# Autodesk Inventor assembly: drive with fourbar linkage
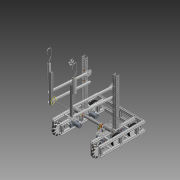
[picture p0: Inventor's stored thumbnail of the model, 180x180]
Saved by Autodesk Inventor 2013 (Build 170138000, 138)
## iProperties
Created: 2013-12-21
Part Number: drive with fourbar linkage
Document SubType Name: Assembly
Designer: kahohbein
Author: kahohbein
## Documents named in this file (22)
- C:\Users\nojessen\Documents\GitHub\2013-2014_BlockParty\CAD\wimp with full update.iam
- C:\Users\nojessen\Documents\GitHub\2013-2014_BlockParty\CAD\Drive\Final Drive Complete\Driveopen2.iam
- C:\Users\nojessen\Documents\GitHub\2013-2014_BlockParty\CAD\COTSParts\Tetrix\Tetrix flat plate.ipt
- C:\Users\nojessen\Documents\GitHub\2013-2014_BlockParty\CAD\COTSParts\Tetrix\Tetrix channel 32mm.ipt
- C:\Users\nojessen\Documents\GitHub\2013-2014_BlockParty\CAD\COTSParts\Tetrix\Bronze bushing.ipt
- C:\Users\nojessen\Documents\GitHub\2013-2014_BlockParty\CAD\COTSParts\Tetrix\Tetrix motor mount.ipt
- C:\Users\nojessen\Documents\GitHub\2013-2014_BlockParty\CAD\Lift\MK3\hook prototype.ipt
- C:\Users\nojessen\Documents\GitHub\2013-2014_BlockParty\CAD\Lift\Bosch 20x20 modified.ipt
- C:\Users\nojessen\Documents\GitHub\2013-2014_BlockParty\CAD\four bar linkage\custom Box Aluminum.ipt
- C:\Users\nojessen\Documents\GitHub\2013-2014_BlockParty\CAD\four bar linkage\custom bosch 8in.ipt
- C:\Users\nojessen\Documents\GitHub\2013-2014_BlockParty\CAD\COTSParts\Tetrix\Tetrix Channel 416mm.ipt
- C:\Users\nojessen\Documents\GitHub\2013-2014_BlockParty\CAD\COTSParts\Tetrix\Tetrix Channel 416mm_CPY.ipt
- C:\Users\nojessen\Documents\GitHub\2013-2014_BlockParty\CAD\COTSParts\Tetrix\Tetrix Hub - axle.ipt
- C:\Users\nojessen\Documents\GitHub\2013-2014_BlockParty\CAD\COTSParts\Tetrix\Tetrix sprocket 24T.ipt
- C:\Users\nojessen\Documents\GitHub\2013-2014_BlockParty\CAD\Lift\MK4\Winch MK4.iam
- C:\Users\nojessen\Documents\GitHub\2013-2014_BlockParty\CAD\COTSParts\Fasteners\4-40 SHCS x125.ipt
- C:\Users\nojessen\Documents\GitHub\2013-2014_BlockParty\CAD\Lift\MK4\ratchet stop mk 2.ipt
- C:\Users\nojessen\Documents\GitHub\2013-2014_BlockParty\CAD\Lift\MK4\Tetrix channel 32mm modified.ipt
- C:\Users\nojessen\Documents\GitHub\2013-2014_BlockParty\CAD\Pick-up Blocks\axle.ipt
- C:\Users\nojessen\Documents\GitHub\2013-2014_BlockParty\CAD\COTSParts\Tetrix\Tetrix sprocket 16T_MIR2.ipt
- C:\Users\nojessen\Documents\GitHub\2013-2014_BlockParty\CAD\COTSParts\Tetrix\Tetrix Hub - axle_MIR2.ipt
- C:\Users\nojessen\Documents\GitHub\2013-2014_BlockParty\CAD\COTSParts\Bosch Extrusion\Gusset 20x20 w screws.ipt
## Components (43 placed, 21 different names)
1. Driveopen2:1 [sub-assembly] — Mate:1, Mate:2, Mate:3, Mate:4, Mate:5, Mate:6
2. Tetrix flat plate:1 — Mate:2, Mate:3, Mate:4, Mate:15, Mate:16, Mate:110, Flush:10, Mate:184, Mate:191, Mate:192, Mate:193, Mate:201, Mate:202
3. Tetrix flat plate:2 — Mate:1, Mate:5, Mate:6, Mate:11, Mate:12, Mate:100, Flush:8, Mate:176, Mate:194, Mate:195, Mate:196, Mate:199, Mate:200
4. Tetrix channel 32mm:1 — Mate:15, Mate:16, Flush:9, Mate:111, Flush:10
5. Tetrix channel 32mm:2 — Mate:11, Mate:12, Mate:101, Flush:7, Flush:8
6. Bronze bushing:6 — Mate:102, Mate:104
7. Bronze bushing:12 — Mate:103, Mate:105
8. hook prototype:1 — Mate:80, Mate:81, Angle:1
9. Bosch 20x20 modified:1 — Mate:80, Mate:81, Mate:99, Flush:6, Flush:11, Angle:1
10. custom Box Aluminum:1 — Flush:5, Mate:96, Mate:148, Mate:151, Mate:152
11. custom Box Aluminum:2 — Flush:4, Mate:97, Mate:140, Mate:143, Mate:144, Mate:145, Mate:146, Mate:147, Mate:206
12. custom Box Aluminum:3 — Flush:5, Mate:134, Mate:155, Mate:156
13. custom Box Aluminum:4 — Flush:4, Mate:124, Mate:126, Mate:129, Mate:130, Mate:131, Mate:135, Mate:207
14. custom bosch 8in:1 — Mate:96, Mate:97, Mate:99, Flush:6, Flush:11, Flush:15, Mate:206, Mate:209, Mate:210
15. Tetrix Channel 416mm:1 — Mate:100, Mate:101, Flush:7, Mate:102, Mate:103, Mate:104, Mate:105, Mate:140, Mate:141, Mate:142, Mate:148, Mate:149, Mate:150
16. Tetrix Channel 416mm_CPY:1 — Mate:110, Flush:9, Mate:111, Mate:132, Mate:133, Mate:153, Mate:154
17. Tetrix Hub - axle:1 — Mate:124, Mate:128, Mate:129, Mate:131, Mate:132, Mate:133
18. Tetrix sprocket 24T:1 — Mate:126, Mate:128, Mate:130
19. custom bosch 8in:2 — Mate:134, Mate:135, Mate:137, Flush:12, Flush:13, Mate:207, Mate:208, Mate:211, Flush:16
20. Bosch 20x20 modified:2 — Mate:137, Flush:12, Flush:13, Mate:138, Mate:139, Angle:2
21. hook prototype:2 — Mate:138, Mate:139, Angle:2
22. Tetrix Hub - axle:2 — Mate:141, Mate:142, Mate:143, Mate:144
23. Tetrix sprocket 24T:2 — Mate:145, Mate:146, Mate:147
24. Tetrix Hub - axle:3 — Mate:149, Mate:150, Mate:151, Mate:152
25. Tetrix Hub - axle:4 — Mate:153, Mate:154, Mate:155, Mate:156
26. Winch MK4:1 [sub-assembly] — Mate:197, Mate:198, Flush:14
27. 4-40 SHCS x125:1 — Mate:179, Mate:181
28. ratchet stop mk 2:1 — Mate:177, Mate:182
29. 4-40 SHCS x125:2 — Mate:178, Mate:180
30. Tetrix channel 32mm modified:1 — Mate:176, Mate:177, Mate:178, Mate:179, Mate:180, Mate:181, Mate:182, Mate:199, Mate:200
31. Tetrix channel 32mm modified:2 — Mate:184, Mate:185, Mate:186, Mate:187, Mate:188, Mate:189, Mate:190, Mate:201, Mate:202
32. ratchet stop mk 2:2 — Mate:187, Mate:188, Flush:14
33. 4-40 SHCS x125:3 — Mate:185, Mate:189
34. 4-40 SHCS x125:4 — Mate:186, Mate:190
35. Tetrix motor mount:1 — Mate:191, Mate:192, Mate:193, Mate:198
36. Tetrix motor mount:2 — Mate:194, Mate:195, Mate:196, Mate:197
37. Bronze bushing:13 — Mate:208, Mate:211, Mate:212
38. Bronze bushing:14 — Mate:209, Mate:210, Mate:217
39. axle:1 — Mate:212, Flush:16, Mate:216
40. Tetrix sprocket 16T_MIR2:1 — Mate:213, Mate:214, Mate:215
41. Tetrix Hub - axle_MIR2:1 — Mate:213, Mate:214, Mate:215, Mate:216, Mate:217
42. Gusset 20x20 w screws:1
43. Gusset 20x20 w screws:2
## Relationships (106: Mate 91, Flush 13, Angle 2)
- Mate:1: Driveopen2:1 ↔ Tetrix flat plate:2
- Mate:2: Driveopen2:1 ↔ Tetrix flat plate:1
- Mate:3 (139.7 mm): Driveopen2:1 ↔ Tetrix flat plate:1
- Mate:4 (63.5 mm): Driveopen2:1 ↔ Tetrix flat plate:1
- Mate:5 (139.7 mm): Driveopen2:1 ↔ Tetrix flat plate:2
- Mate:6 (63.5 mm): Driveopen2:1 ↔ Tetrix flat plate:2
- Mate:11: Tetrix flat plate:2 ↔ Tetrix channel 32mm:2
- Mate:12: Tetrix flat plate:2 ↔ Tetrix channel 32mm:2
- Mate:15: Tetrix flat plate:1 ↔ Tetrix channel 32mm:1
- Mate:16: Tetrix flat plate:1 ↔ Tetrix channel 32mm:1
- Mate:80: hook prototype:1 ↔ Bosch 20x20 modified:1
- Mate:81: hook prototype:1 ↔ Bosch 20x20 modified:1
- Flush:4: custom Box Aluminum:2 ↔ custom Box Aluminum:4
- Flush:5: custom Box Aluminum:1 ↔ custom Box Aluminum:3
- Mate:96: custom Box Aluminum:1 ↔ custom bosch 8in:1
- Mate:97: custom Box Aluminum:2 ↔ custom bosch 8in:1
- Mate:99: Bosch 20x20 modified:1 ↔ custom bosch 8in:1
- Flush:6: Bosch 20x20 modified:1 ↔ custom bosch 8in:1
- Mate:100: Tetrix flat plate:2 ↔ Tetrix Channel 416mm:1
- Mate:101: Tetrix channel 32mm:2 ↔ Tetrix Channel 416mm:1
- Flush:7: Tetrix channel 32mm:2 ↔ Tetrix Channel 416mm:1
- Flush:8: Tetrix flat plate:2 ↔ Tetrix channel 32mm:2
- Mate:102: Bronze bushing:6 ↔ Tetrix Channel 416mm:1
- Mate:103: Bronze bushing:12 ↔ Tetrix Channel 416mm:1
- Mate:104: Bronze bushing:6 ↔ Tetrix Channel 416mm:1
- Mate:105: Bronze bushing:12 ↔ Tetrix Channel 416mm:1
- Mate:110: Tetrix flat plate:1 ↔ Tetrix Channel 416mm_CPY:1
- Flush:9: Tetrix channel 32mm:1 ↔ Tetrix Channel 416mm_CPY:1
- Mate:111: Tetrix channel 32mm:1 ↔ Tetrix Channel 416mm_CPY:1
- Flush:10: Tetrix flat plate:1 ↔ Tetrix channel 32mm:1
- Flush:11 (60.833 mm): Bosch 20x20 modified:1 ↔ custom bosch 8in:1
- Mate:124: custom Box Aluminum:4 ↔ Tetrix Hub - axle:1
- Mate:126: custom Box Aluminum:4 ↔ Tetrix sprocket 24T:1
- Mate:128: Tetrix Hub - axle:1 ↔ Tetrix sprocket 24T:1
- Mate:129: custom Box Aluminum:4 ↔ Tetrix Hub - axle:1
- Mate:130: custom Box Aluminum:4 ↔ Tetrix sprocket 24T:1
- Mate:131: custom Box Aluminum:4 ↔ Tetrix Hub - axle:1
- Mate:132: Tetrix Channel 416mm_CPY:1 ↔ Tetrix Hub - axle:1
- Mate:133: Tetrix Channel 416mm_CPY:1 ↔ Tetrix Hub - axle:1
- Mate:134: custom Box Aluminum:3 ↔ custom bosch 8in:2
- Mate:135: custom Box Aluminum:4 ↔ custom bosch 8in:2
- Mate:137: custom bosch 8in:2 ↔ Bosch 20x20 modified:2
- Flush:12: custom bosch 8in:2 ↔ Bosch 20x20 modified:2
- Flush:13 (-60.833 mm): custom bosch 8in:2 ↔ Bosch 20x20 modified:2
- Mate:138: Bosch 20x20 modified:2 ↔ hook prototype:2
- Mate:139 (-15.24 mm): Bosch 20x20 modified:2 ↔ hook prototype:2
- Mate:140: custom Box Aluminum:2 ↔ Tetrix Channel 416mm:1
- Mate:141: Tetrix Channel 416mm:1 ↔ Tetrix Hub - axle:2
- Mate:142: Tetrix Channel 416mm:1 ↔ Tetrix Hub - axle:2
- Mate:143: custom Box Aluminum:2 ↔ Tetrix Hub - axle:2
- Mate:144: custom Box Aluminum:2 ↔ Tetrix Hub - axle:2
- Mate:145: custom Box Aluminum:2 ↔ Tetrix sprocket 24T:2
- Mate:146: custom Box Aluminum:2 ↔ Tetrix sprocket 24T:2
- Mate:147: custom Box Aluminum:2 ↔ Tetrix sprocket 24T:2
- Mate:148: custom Box Aluminum:1 ↔ Tetrix Channel 416mm:1
- Mate:149: Tetrix Channel 416mm:1 ↔ Tetrix Hub - axle:3
- Mate:150: Tetrix Channel 416mm:1 ↔ Tetrix Hub - axle:3
- Mate:151: custom Box Aluminum:1 ↔ Tetrix Hub - axle:3
- Mate:152: custom Box Aluminum:1 ↔ Tetrix Hub - axle:3
- Mate:153: Tetrix Channel 416mm_CPY:1 ↔ Tetrix Hub - axle:4
- Mate:154: Tetrix Channel 416mm_CPY:1 ↔ Tetrix Hub - axle:4
- Mate:155: custom Box Aluminum:3 ↔ Tetrix Hub - axle:4
- Mate:156: custom Box Aluminum:3 ↔ Tetrix Hub - axle:4
- Mate:176: Tetrix flat plate:2 ↔ Tetrix channel 32mm modified:1
- Mate:177: ratchet stop mk 2:1 ↔ Tetrix channel 32mm modified:1
- Mate:178: 4-40 SHCS x125:2 ↔ Tetrix channel 32mm modified:1
- Mate:179: 4-40 SHCS x125:1 ↔ Tetrix channel 32mm modified:1
- Mate:180: 4-40 SHCS x125:2 ↔ Tetrix channel 32mm modified:1
- Mate:181: 4-40 SHCS x125:1 ↔ Tetrix channel 32mm modified:1
- Mate:182: ratchet stop mk 2:1 ↔ Tetrix channel 32mm modified:1
- Mate:184: Tetrix flat plate:1 ↔ Tetrix channel 32mm modified:2
- Mate:185: Tetrix channel 32mm modified:2 ↔ 4-40 SHCS x125:3
- Mate:186: Tetrix channel 32mm modified:2 ↔ 4-40 SHCS x125:4
- Mate:187: Tetrix channel 32mm modified:2 ↔ ratchet stop mk 2:2
- Mate:188: Tetrix channel 32mm modified:2 ↔ ratchet stop mk 2:2
- Mate:189: Tetrix channel 32mm modified:2 ↔ 4-40 SHCS x125:3
- Mate:190: Tetrix channel 32mm modified:2 ↔ 4-40 SHCS x125:4
- Mate:191: Tetrix flat plate:1 ↔ Tetrix motor mount:1
- Mate:192: Tetrix flat plate:1 ↔ Tetrix motor mount:1
- Mate:193: Tetrix flat plate:1 ↔ Tetrix motor mount:1
- Mate:194: Tetrix flat plate:2 ↔ Tetrix motor mount:2
- Mate:195: Tetrix flat plate:2 ↔ Tetrix motor mount:2
- Mate:196: Tetrix flat plate:2 ↔ Tetrix motor mount:2
- Mate:197: Winch MK4:1 ↔ Tetrix motor mount:2
- Mate:198: Winch MK4:1 ↔ Tetrix motor mount:1
- Mate:199: Tetrix flat plate:2 ↔ Tetrix channel 32mm modified:1
- Mate:200: Tetrix flat plate:2 ↔ Tetrix channel 32mm modified:1
- Mate:201: Tetrix flat plate:1 ↔ Tetrix channel 32mm modified:2
- Mate:202: Tetrix flat plate:1 ↔ Tetrix channel 32mm modified:2
- Flush:14: Winch MK4:1 ↔ ratchet stop mk 2:2
- Angle:1 (90 deg): hook prototype:1 ↔ Bosch 20x20 modified:1
- Angle:2 (90 deg): Bosch 20x20 modified:2 ↔ hook prototype:2
- Flush:15 (85.9981 mm): custom bosch 8in:1
- Mate:206: custom Box Aluminum:2 ↔ custom bosch 8in:1
- Mate:207: custom Box Aluminum:4 ↔ custom bosch 8in:2
- Mate:208: custom bosch 8in:2 ↔ Bronze bushing:13
- Mate:209: custom bosch 8in:1 ↔ Bronze bushing:14
- Mate:210: custom bosch 8in:1 ↔ Bronze bushing:14
- Mate:211: custom bosch 8in:2 ↔ Bronze bushing:13
- Mate:212: Bronze bushing:13 ↔ axle:1
- Flush:16 (-17.8308 mm): custom bosch 8in:2 ↔ axle:1
- Mate:213: Tetrix sprocket 16T_MIR2:1 ↔ Tetrix Hub - axle_MIR2:1
- Mate:214: Tetrix sprocket 16T_MIR2:1 ↔ Tetrix Hub - axle_MIR2:1
- Mate:215: Tetrix sprocket 16T_MIR2:1 ↔ Tetrix Hub - axle_MIR2:1
- Mate:216: axle:1 ↔ Tetrix Hub - axle_MIR2:1
- Mate:217 (3.175 mm): Bronze bushing:14 ↔ Tetrix Hub - axle_MIR2:1
